# Autodesk Inventor assembly: Leafers_MIR
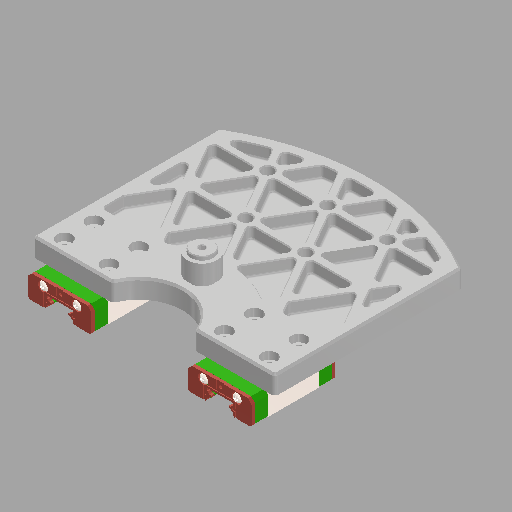
[picture p0: Inventor's stored thumbnail of the model, 512x512]
Saved by Autodesk Inventor 2027 (Build 310192060, 192F)
## iProperties
Created: 2026-06-26
Part Number: Leafers_MIR
Document SubType Name: Assembly
Designer: opore
Author: opore
## Documents named in this file (4)
- H:\Autodesk\AirBrake\AirBrakeReal\Leafers_MIR.iam
- H:\Autodesk\AirBrake\AirBrakeReal\_CFFANG4-8_1_MIR.ipt
- H:\Autodesk\AirBrake\AirBrakeReal\Leaf 2_MIR1.ipt
- H:\Autodesk\AirBrake\AirBrakeReal\MGN7C\MGN7C_MIR.ipt
## Components (4 placed, 3 different names)
1. _CFFANG4-8_1_MIR:1 — Rotational:1
2. Leaf 2_MIR1:1 — Rotational:1, Rigid:1, Rotational:2
3. MGN7C_MIR:1 — Rigid:1
4. MGN7C_MIR:2 — Rotational:2
## Relationships (3: RevoluteJoint 2, WeldJoint 1)
- Rotational:1 [RevoluteJoint]: _CFFANG4-8_1_MIR:1 ↔ Leaf 2_MIR1:1
- Rigid:1 [WeldJoint]: Leaf 2_MIR1:1 ↔ MGN7C_MIR:1
- Rotational:2 [RevoluteJoint]: Leaf 2_MIR1:1 ↔ MGN7C_MIR:2
